# Autodesk Inventor assembly: Assembly1
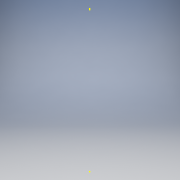
[picture p0: Inventor's stored thumbnail of the model, 180x180]
Saved by Autodesk Inventor 2019 (Build 230136000, 136)
## iProperties
Created: 2020-03-04
Part Number: Assembly1
Document SubType Name: Assembly
Designer: Dell
Author: Dell
## Documents named in this file (5)
- F:\self balancing bot\Assembly1.iam
- F:\virtual implementation new\bodyyyyyyyyyy.ipt
- F:\virtual implementation new\clamp.ipt
- F:\exploration virtual\head_MIR.ipt
- F:\exploration virtual\new robo wheel.ipt
## Components (6 placed, 4 different names)
1. bodyyyyyyyyyy:1 — Mate:1, Mate:2, Rigid:3, Mate:3, Rotational:1, Rotational:2
2. clamp:3 — Mate:2, Mate:3
3. clamp:6 — Mate:1
4. head_MIR:1 — Rigid:3
5. new robo wheel:1 — Rotational:2
6. new robo wheel:2 — Rotational:1
## Relationships (6: Mate 3, RevoluteJoint 2, WeldJoint 1)
- Mate:1: bodyyyyyyyyyy:1 ↔ clamp:6
- Mate:2: bodyyyyyyyyyy:1 ↔ clamp:3
- Rigid:3 [WeldJoint]: bodyyyyyyyyyy:1 ↔ head_MIR:1
- Mate:3: bodyyyyyyyyyy:1 ↔ clamp:3
- Rotational:1 [RevoluteJoint]: bodyyyyyyyyyy:1 ↔ new robo wheel:2
- Rotational:2 [RevoluteJoint]: bodyyyyyyyyyy:1 ↔ new robo wheel:1
